# Autodesk Inventor assembly: femur + horn
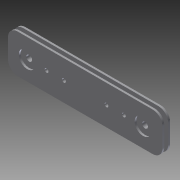
[picture p0: Inventor's stored thumbnail of the model, 180x180]
Saved by Autodesk Inventor 2012 (Build 160160000, 160)
## iProperties
Created: 2013-12-06
Part Number: femur + horn
Document SubType Name: Assembly
Designer: Irwan Haryanto
Author: Irwan Haryanto
## Documents named in this file (3)
- D:\Revenant\robot baru 2014\femur + horn.iam
- D:\Revenant\robot baru 2014\sketch femur 6 cm.ipt
- D:\Revenant\robot baru 2014\Horn.ipt
## Components (4 placed, 2 different names)
1. sketch femur 6 cm:1 — Insert:5, Insert:6
2. sketch femur 6 cm:2 — Insert:1, Insert:2, Insert:3, Insert:4
3. Horn:1 — Insert:2, Insert:4, Insert:6
4. Horn:2 — Insert:1, Insert:3, Insert:5
## Relationships (6: Insert 6)
- Insert:1: sketch femur 6 cm:2 ↔ Horn:2
- Insert:2: sketch femur 6 cm:2 ↔ Horn:1
- Insert:3: sketch femur 6 cm:2 ↔ Horn:2
- Insert:4: sketch femur 6 cm:2 ↔ Horn:1
- Insert:5: sketch femur 6 cm:1 ↔ Horn:2
- Insert:6: sketch femur 6 cm:1 ↔ Horn:1
